# Autodesk Inventor assembly: HeadBarClamp
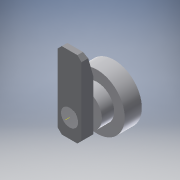
[picture p0: Inventor's stored thumbnail of the model, 180x180]
Saved by Autodesk Inventor 2016 (Build 200138000, 138)
## iProperties
Created: 2015-11-18
Part Number: HeadBarClamp
Document SubType Name: Assembly
Designer: Vervaeke-Lab
Author: Vervaeke-Lab
## Documents named in this file (4)
- C:\Users\Vervaeke-Lab\Desktop\inventor\inventor_parts\HeadBarClamp.iam
- C:\Users\Vervaeke-Lab\Desktop\inventor\inventor_parts\HeadbarClamp.ipt
- C:\Users\Vervaeke-Lab\Desktop\inventor\inventor_parts\HeadBarClampScrew.ipt
- C:\Users\Vervaeke-Lab\Desktop\inventor\inventor_parts\HeadBarClampTurnwheel.ipt
## Components (3 placed, 3 different names)
1. HeadbarClamp:1 — Mate:1, Flush:1
2. HeadBarClampScrew:1 — Mate:1, Flush:1, Mate:2, Flush:2
3. HeadBarClampTurnwheel:1 — Mate:2, Flush:2
## Relationships (4: Mate 2, Flush 2)
- Mate:1: HeadbarClamp:1 ↔ HeadBarClampScrew:1
- Flush:1: HeadbarClamp:1 ↔ HeadBarClampScrew:1
- Mate:2: HeadBarClampScrew:1 ↔ HeadBarClampTurnwheel:1
- Flush:2: HeadBarClampScrew:1 ↔ HeadBarClampTurnwheel:1
